# Autodesk Inventor assembly: vp13
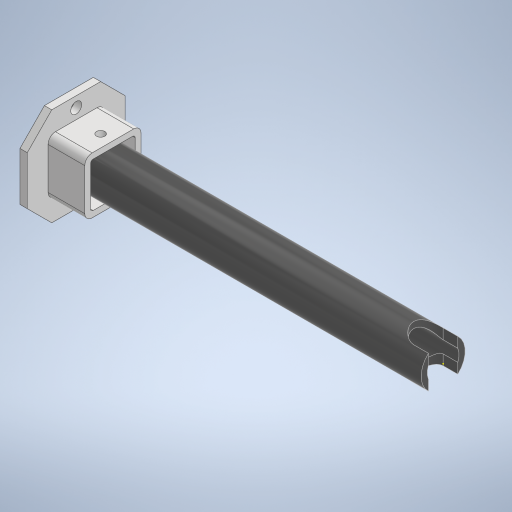
[picture p0: Inventor's stored thumbnail of the model, 512x512]
Saved by Autodesk Inventor 2024 (Build 280153000, 153)
## iProperties
Created: 2025-05-23
Part Number: vp13
Document SubType Name: Assembly
Designer: 1412z
Author: 1412z
## Documents named in this file (3)
- C:\Users\1412z\OneDrive\デスクトップ\rdclab\harvesting_robot\harvesting_endeffector\demo_rod_endeffector\vp13.iam
- C:\Users\1412z\OneDrive\デスクトップ\rdclab\harvesting_robot\harvesting_endeffector\demo_rod_endeffector\vp13_150.ipt
- C:\Users\1412z\OneDrive\デスクトップ\rdclab\harvesting_robot\harvesting_endeffector\demo_rod_endeffector\rod_fixture_vp13.ipt
## Components (2 placed, 2 different names)
1. vp13_150:1 — 回転:1
2. rod_fixture_vp13:1 — 回転:1
## Relationships (1: RevoluteJoint 1)
- 回転:1 [RevoluteJoint]: vp13_150:1 ↔ rod_fixture_vp13:1
